# Autodesk Inventor assembly: 5SS_Platform
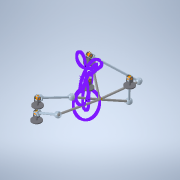
[picture p0: Inventor's stored thumbnail of the model, 180x180]
Saved by Autodesk Inventor 2020.1 (Build 241239000, 239)
## iProperties
Created: 2019-10-24
Part Number: 5SS_Platform
Document SubType Name: Assembly
Designer: sshel
Author: sshel
## Documents named in this file (13)
- D:\Desktop 2019\MS, Phd\Sem8- 2019 Spring (RA, 3research)\Spatial approach- Spherical and Planar synthesis\CAD\5US Platform\5US_Platform.iam
- D:\Desktop 2019\MS, Phd\Sem8- 2019 Spring (RA, 3research)\Spatial approach- Spherical and Planar synthesis\CAD\5US Platform\Components\U_FP.ipt
- D:\Desktop 2019\MS, Phd\Sem8- 2019 Spring (RA, 3research)\Spatial approach- Spherical and Planar synthesis\CAD\5US Platform\Components\Coupler.ipt
- D:\Desktop 2019\MS, Phd\Sem8- 2019 Spring (RA, 3research)\Spatial approach- Spherical and Planar synthesis\CAD\5US Platform\Components\US_Dyad.ipt
- D:\Desktop 2019\MS, Phd\Sem8- 2019 Spring (RA, 3research)\Spatial approach- Spherical and Planar synthesis\CAD\5US Platform\Components\U_Joint_Center.ipt
- D:\Desktop 2019\MS, Phd\Sem8- 2019 Spring (RA, 3research)\Spatial approach- Spherical and Planar synthesis\CAD\5US Platform\Components\US_Dyad\US_Dyad-01.ipt
- D:\Desktop 2019\MS, Phd\Sem8- 2019 Spring (RA, 3research)\Spatial approach- Spherical and Planar synthesis\CAD\5US Platform\Components\US_Dyad\US_Dyad-02.ipt
- D:\Desktop 2019\MS, Phd\Sem8- 2019 Spring (RA, 3research)\Spatial approach- Spherical and Planar synthesis\CAD\5US Platform\Components\US_Dyad\US_Dyad-03.ipt
- D:\Desktop 2019\MS, Phd\Sem8- 2019 Spring (RA, 3research)\Spatial approach- Spherical and Planar synthesis\CAD\5US Platform\Components\US_Dyad\US_Dyad-04.ipt
- D:\Desktop 2019\MS, Phd\Sem8- 2019 Spring (RA, 3research)\Spatial approach- Spherical and Planar synthesis\CAD\5US Platform\Components\US_Dyad\US_Dyad-05.ipt
- D:\Desktop 2019\MS, Phd\Sem8- 2019 Spring (RA, 3research)\Spatial approach- Spherical and Planar synthesis\CAD\5US Platform\Components\Coupler_Paths.ipt
- D:\Desktop 2019\MS, Phd\Sem8- 2019 Spring (RA, 3research)\Spatial approach- Spherical and Planar synthesis\CAD\5US Platform\Components\Poses.ipt
- D:\Desktop 2019\MS, Phd\Sem8- 2019 Spring (RA, 3research)\Spatial approach- Spherical and Planar synthesis\CAD\5US Platform\Linked Parameters.xlsx
## Components (18 placed, 10 different names)
1. U_FP:1 — Flush:3, Rotational:1
2. U_FP:2 — Flush:6, Rotational:2
3. U_FP:3 — Flush:9, Rotational:3
4. U_FP:4 — Flush:12, Rotational:4
5. U_FP:5 — Flush:15, Rotational:5
6. Coupler:1 — Ball:1, Ball:2, Ball:3, Ball:4, Ball:5
7. U_Joint_Center:1 — Rotational:1, Rotational:6
8. U_Joint_Center:2 — Rotational:2, Rotational:7
9. U_Joint_Center:3 — Rotational:3, Rotational:8
10. U_Joint_Center:4 — Rotational:4, Rotational:9
11. U_Joint_Center:5 — Rotational:5, Rotational:10
12. US_Dyad-01:1 — Rotational:6, Ball:1
13. US_Dyad-02:2 — Rotational:7, Ball:2
14. US_Dyad-03:3 — Rotational:8, Ball:3
15. US_Dyad-04:4 — Rotational:9, Ball:4
16. US_Dyad-05:5 — Rotational:10, Ball:5
17. Coupler_Paths:1
18. Poses
## Relationships (30: Flush 15, RevoluteJoint 10, BallJoint 5)
- [Flush]: U_FP:1
- [Flush]: U_FP:1
- Flush:3: U_FP:1
- [Flush]: U_FP:2
- [Flush]: U_FP:2
- Flush:6: U_FP:2
- [Flush]: U_FP:3
- [Flush]: U_FP:3
- Flush:9: U_FP:3
- [Flush]: U_FP:4
- [Flush]: U_FP:4
- Flush:12: U_FP:4
- [Flush]: U_FP:5
- [Flush]: U_FP:5
- Flush:15: U_FP:5
- Rotational:1 [RevoluteJoint]: U_FP:1 ↔ U_Joint_Center:1
- Rotational:2 [RevoluteJoint]: U_FP:2 ↔ U_Joint_Center:2
- Rotational:3 [RevoluteJoint]: U_FP:3 ↔ U_Joint_Center:3
- Rotational:4 [RevoluteJoint]: U_FP:4 ↔ U_Joint_Center:4
- Rotational:5 [RevoluteJoint]: U_FP:5 ↔ U_Joint_Center:5
- Rotational:6 [RevoluteJoint]: U_Joint_Center:1 ↔ US_Dyad-01:1
- Rotational:7 [RevoluteJoint]: U_Joint_Center:2 ↔ US_Dyad-02:2
- Rotational:8 [RevoluteJoint]: U_Joint_Center:3 ↔ US_Dyad-03:3
- Rotational:9 [RevoluteJoint]: U_Joint_Center:4 ↔ US_Dyad-04:4
- Rotational:10 [RevoluteJoint]: U_Joint_Center:5 ↔ US_Dyad-05:5
- Ball:1: Coupler:1 ↔ US_Dyad-01:1
- Ball:2: Coupler:1 ↔ US_Dyad-02:2
- Ball:3: Coupler:1 ↔ US_Dyad-03:3
- Ball:4: Coupler:1 ↔ US_Dyad-04:4
- Ball:5: Coupler:1 ↔ US_Dyad-05:5
## Named parameters: dyad1_Fx = -4260.66351 mm, dyad1_Fy = 914.69194 mm, dyad1_Fz = 2675.35545 mm, dyad5_Fy = -2032.16374 mm, dyad5_Fx = 3055.55556 mm, dyad5_Fz = 2423.97661 mm, dyad4_Fz = 2764.89028 mm, dyad4_Fy = 2100.31348 mm, dyad4_Fx = 2692.78997 mm, dyad3_Fz = 1248 mm, dyad3_Fx = -4318 mm, dyad2_Fz = 3417.84038 mm, dyad3_Fy = 970 mm, dyad2_Fx = -451.87793 mm, dyad2_Fy = -915.49296 mm, L1 = 2975.73867 mm, L2 = 2688.57306 mm, L3 = 2779.3532 mm, L4 = 4651.10383 mm, L5 = 3279.55138 mm
